# Autodesk Inventor assembly: proxima_kicadproxima_sensor_board
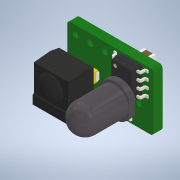
[picture p0: Inventor's stored thumbnail of the model, 180x180]
Saved by Autodesk Inventor 2021 (Build 250183000, 183)
## iProperties
Company: A Company
Created: 2021-08-02
Part Number: proxima_kicadproxima_sensor_board
Description: KiCad electronic assembly
Document SubType Name: Assembly
Designer: ermoz
Authority: Unknown
Sending System: KiCad to STEP converter
Preprocessor: Open CASCADE STEP processor 6.9
Title: proxima_sensor_board.step
Author: An Author
## Documents named in this file (9)
- D:\Moje Wyczyny\My_Poor_Projects\Proxima_sensor\proxima-sensor\version_1.xx\proxima_sensor_case\exported_from_kicad\proxima_kicadproxima_sensor_board.iam
- D:\Moje Wyczyny\My_Poor_Projects\Proxima_sensor\proxima-sensor\version_1.xx\proxima_sensor_case\exported_from_kicad\proxima_kicadCP_EIA-3216-10_Kemet-I.iam
- D:\Moje Wyczyny\My_Poor_Projects\Proxima_sensor\proxima-sensor\version_1.xx\proxima_sensor_case\exported_from_kicad\proxima_kicadSOIC-8_3.9x4.9mm_P1.27mm.iam
- D:\Moje Wyczyny\My_Poor_Projects\Proxima_sensor\proxima-sensor\version_1.xx\proxima_sensor_case\exported_from_kicad\proxima_kicadVishay_MOLD-3Pin.iam
- D:\Moje Wyczyny\My_Poor_Projects\Proxima_sensor\proxima-sensor\version_1.xx\proxima_sensor_case\exported_from_kicad\proxima_kicadR_0805_2012Metric.iam
- D:\Moje Wyczyny\My_Poor_Projects\Proxima_sensor\proxima-sensor\version_1.xx\proxima_sensor_case\exported_from_kicad\proxima_kicadLED_0805_2012Metric.iam
- D:\Moje Wyczyny\My_Poor_Projects\Proxima_sensor\proxima-sensor\version_1.xx\proxima_sensor_case\exported_from_kicad\proxima_kicadLED_D5.0mm_IRGrey.iam
- D:\Moje Wyczyny\My_Poor_Projects\Proxima_sensor\proxima-sensor\version_1.xx\proxima_sensor_case\exported_from_kicad\proxima_kicadC_0805_2012Metric.iam
- D:\Moje Wyczyny\My_Poor_Projects\Proxima_sensor\proxima-sensor\version_1.xx\proxima_sensor_case\exported_from_kicad\proxima_kicadCOMPOUND.ipt
## Components (13 placed, 13 different names)
1. 4 [sub-assembly] — Mate:1
2. 6 [sub-assembly]
3. 8 [sub-assembly] — Mate:1
4. 10 [sub-assembly]
5. 11 [sub-assembly]
6. 12 [sub-assembly]
7. 13 [sub-assembly]
8. 14 [sub-assembly]
9. 16 [sub-assembly]
10. 18 [sub-assembly] — Mate:2, Mate:3, Angle:1
11. 20 [sub-assembly]
12. 21 [sub-assembly]
13. 22 — Mate:2, Mate:3, Angle:1
## Relationships (4: Mate 3, Angle 1)
- Mate:1 (1 mm): 4 ↔ 8
- Mate:2 (2 mm): 18 ↔ 22
- Mate:3 (-5 mm): 18 ↔ 22
- Angle:1 (0 deg): 18 ↔ 22
